# Autodesk Inventor assembly: Assembly1
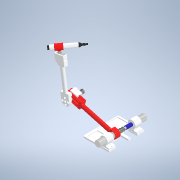
[picture p0: Inventor's stored thumbnail of the model, 180x180]
Saved by Autodesk Inventor 2021 (Build 250183000, 183)
## iProperties
Created: 2022-11-17
Part Number: Assembly1
Document SubType Name: Assembly
Designer: zulet
Author: zulet
## Documents named in this file (5)
- D:\UNAL\2022-2S\Servomecanismos\Proyecto Academico\SImscape\Assembly1.iam
- D:\UNAL\2022-2S\Servomecanismos\Proyecto Academico\SImscape\sim_BASE.ipt
- D:\UNAL\2022-2S\Servomecanismos\Proyecto Academico\SImscape\sim_LINK1.ipt
- D:\UNAL\2022-2S\Servomecanismos\Proyecto Academico\SImscape\sim_LINK2.ipt
- D:\UNAL\2022-2S\Servomecanismos\Proyecto Academico\SImscape\sim_MARCADOR.ipt
## Components (4 placed, 4 different names)
1. sim_LINK1:1 — Mate:1, Mate:2, Mate:3, Mate:4
2. sim_MARCADOR:1 — Mate:5, Mate:6
3. sim_BASE:1 — Mate:1, Mate:2
4. sim_LINK2:1 — Mate:3, Mate:4, Mate:5, Mate:6
## Relationships (6: Mate 6)
- Mate:1: sim_LINK1:1 ↔ sim_BASE:1
- Mate:2: sim_LINK1:1 ↔ sim_BASE:1
- Mate:3: sim_LINK1:1 ↔ sim_LINK2:1
- Mate:4 (3 mm): sim_LINK1:1 ↔ sim_LINK2:1
- Mate:5: sim_MARCADOR:1 ↔ sim_LINK2:1
- Mate:6: sim_MARCADOR:1 ↔ sim_LINK2:1
